# Autodesk Inventor assembly: писюны_MIR1
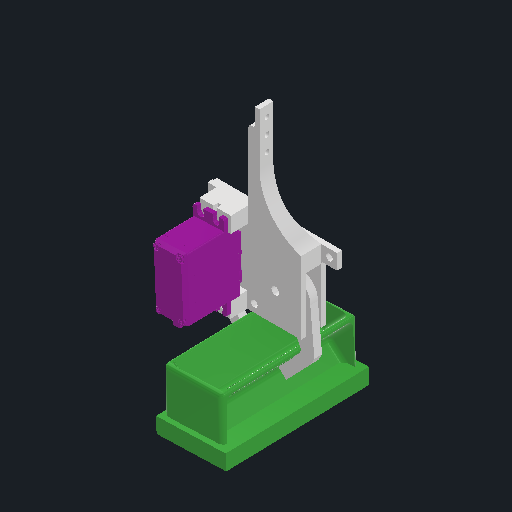
[picture p0: Inventor's stored thumbnail of the model, 512x512]
Saved by Autodesk Inventor 2025 (Build 290162000, 162)
## iProperties
Created: 2024-12-28
Part Number: писюны_MIR1
Document SubType Name: Assembly
Designer: GameHD
Author: Phantom
## Documents named in this file (8)
- C:\Users\GameHD\Desktop\phantom 16950\писюны_MIR1.iam
- C:\Users\GameHD\Desktop\phantom 16950\am-5401 Sample_MIR1_MIR.ipt
- C:\Users\GameHD\Desktop\phantom 16950\2000-0025-0002\2000-0025-0002_MIR4_MIR.ipt
- C:\Users\GameHD\Downloads\Telegram Desktop\tetrix_metal_servo_horn\tetrix_metal_servo_horn_MIR.ipt
- C:\Users\GameHD\Desktop\phantom 16950\держать писюны_MIR1.ipt
- C:\Users\GameHD\Desktop\phantom 16950\писюн 2_MIR3.ipt
- C:\Users\GameHD\Desktop\phantom 16950\писюн_MIR1.ipt
- C:\Users\GameHD\Desktop\phantom 16950\держать писюны 2ч_MIR.ipt
## Components (7 placed, 7 different names)
1. am-5401 Sample_MIR1_MIR:1 — Совмещение:24, Совмещение:23
2. 2000-0025-0002_MIR4_MIR:1 — Совмещение:11, Совмещение:10, Совмещение:17
3. tetrix_metal_servo_horn_MIR:1 — Совмещение:11, Совмещение:10, Совмещение:16, Совмещение:18, Совмещение:19, Совмещение:15
4. держать писюны_MIR1:1 — Совмещение:17, Совмещение:16, Заподлицо:1, Совмещение:22
5. писюн 2_MIR3:1 — Совмещение:24, Совмещение:18
6. писюн_MIR1:1 — Совмещение:23, Совмещение:19, Совмещение:15, Совмещение:21
7. держать писюны 2ч_MIR:1 — Заподлицо:1, Совмещение:22, Совмещение:21
## Relationships (12: Mate 11, Flush 1)
- Совмещение:11 [Mate]: 2000-0025-0002_MIR4_MIR:1 ↔ tetrix_metal_servo_horn_MIR:1
- Совмещение:10 [Mate]: 2000-0025-0002_MIR4_MIR:1 ↔ tetrix_metal_servo_horn_MIR:1
- Совмещение:17 [Mate]: 2000-0025-0002_MIR4_MIR:1 ↔ держать писюны_MIR1:1
- Совмещение:16 [Mate]: tetrix_metal_servo_horn_MIR:1 ↔ держать писюны_MIR1:1
- Совмещение:24 [Mate]: am-5401 Sample_MIR1_MIR:1 ↔ писюн 2_MIR3:1
- Совмещение:18 [Mate]: tetrix_metal_servo_horn_MIR:1 ↔ писюн 2_MIR3:1
- Совмещение:23 [Mate]: am-5401 Sample_MIR1_MIR:1 ↔ писюн_MIR1:1
- Совмещение:19 [Mate]: tetrix_metal_servo_horn_MIR:1 ↔ писюн_MIR1:1
- Совмещение:15 [Mate]: tetrix_metal_servo_horn_MIR:1 ↔ писюн_MIR1:1
- Заподлицо:1 [Flush]: держать писюны_MIR1:1 ↔ держать писюны 2ч_MIR:1
- Совмещение:22 [Mate]: держать писюны_MIR1:1 ↔ держать писюны 2ч_MIR:1
- Совмещение:21 [Mate]: писюн_MIR1:1 ↔ держать писюны 2ч_MIR:1
